# Autodesk Inventor assembly: teljes2
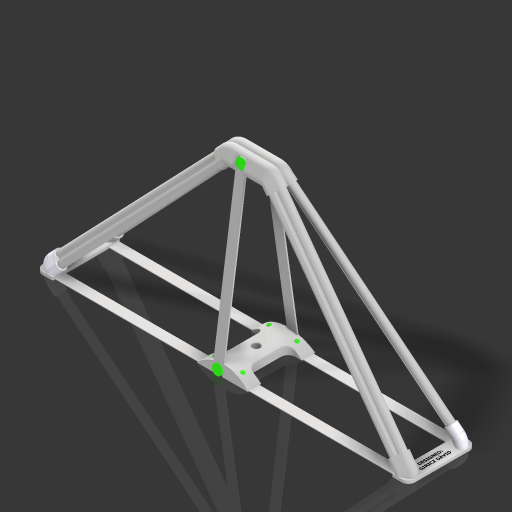
[picture p0: Inventor's stored thumbnail of the model, 512x512]
Saved by Autodesk Inventor 2023 (Build 270158000, 158)
## iProperties
Created: 2022-11-11
Part Number: teljes2
Document SubType Name: Assembly
Designer: gd1
Author: gd1
## Documents named in this file (7)
- C:\Users\gd1\3D Objects\3D nagyteherbírású híd\Híd\H-d\teljes2.iam
- C:\Users\gd1\3D Objects\3D nagyteherbírású híd\Híd\H-d\teljes3.iam
- C:\Users\gd1\3D Objects\3D nagyteherbírású híd\Híd\H-d\teljes4.iam
- C:\Users\gd1\3D Objects\3D nagyteherbírású híd\Híd\H-d\teljes2\AIP\FEA\e5f3hmjog.fins
- C:\Users\gd1\3D Objects\3D nagyteherbírású híd\Híd\H-d\teljes2\AIP\FEA\e5f3hmjpc.fsat
- C:\Users\gd1\3D Objects\3D nagyteherbírású híd\Híd\H-d\teljes2\AIP\FEA\e5f3hmjpc.ftes
- C:\Users\gd1\3D Objects\3D nagyteherbírású híd\Híd\H-d\teljes2\AIP\FEA\e5f3hmjq8.fwiz
## Components (2 placed, 2 different names)
1. teljes4:2 [sub-assembly] — Rigid:1
2. teljes3:1 [sub-assembly] — Rigid:1
## Relationships (1: WeldJoint 1)
- Rigid:1 [WeldJoint]: teljes4:2 ↔ teljes3:1
## Named parameters: sa_0 = 50000
note: some values were not read from the file. Shown as the stored number, unit unknown: "sa_0".
